# Autodesk Inventor assembly: ASM Printing Head
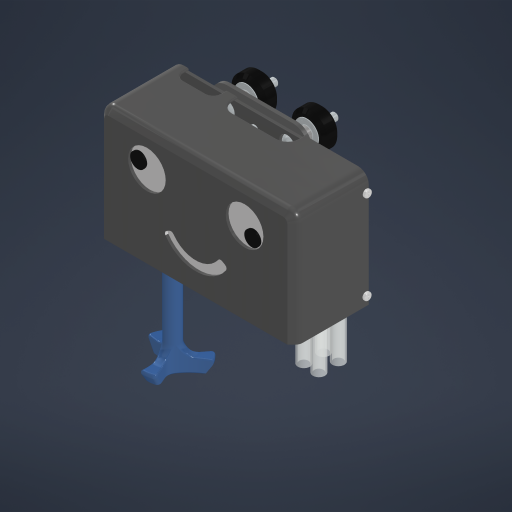
[picture p0: Inventor's stored thumbnail of the model, 512x512]
Saved by Autodesk Inventor 2024 (Build 280153000, 153)
## iProperties
Created: 2018-08-15
Part Number: ASM Printing Head
Document SubType Name: Assembly
Designer: Vincent Larson
Author: Vincent Larson
## Documents named in this file (13)
- C:\Users\Vincent Larson\Downloads\Ender-3 Parts\01 MAIN ASM Ender_3\ASM Printing Head.iam
- C:\Users\Vincent Larson\Downloads\Ender-3 Parts\01 MAIN ASM Ender_3\E plate.ipt
- C:\Users\Vincent Larson\Downloads\Ender-3 Parts\01 MAIN ASM Ender_3\ASM Roller X-Axis.iam
- C:\Users\Vincent Larson\Downloads\Ender-3 Parts\01 MAIN ASM Ender_3\ASM Eccentrical Roller X-Axis.iam
- C:\Users\Vincent Larson\Downloads\Ender-3 Parts\01 MAIN ASM Ender_3\M3X6Pan Head Screw.ipt
- C:\Users\Vincent Larson\Downloads\Motor Bracket.ipt
- C:\Users\Vincent Larson\Downloads\Shaft.ipt
- C:\Users\Vincent Larson\Downloads\Mixing Motor.ipt
- C:\Users\Vincent Larson\Downloads\Tubing.ipt
- C:\Users\Vincent Larson\Downloads\Control Box - Screw.ipt
- C:\Users\Vincent Larson\Downloads\Paper piece.ipt
- C:\Users\Vincent Larson\Downloads\eye.ipt
- C:\Users\Vincent Larson\Downloads\Mixer and nozzle cover.ipt
## Components (24 placed, 12 different names)
1. E plate:1 — Mate:16, Mate:17, Mate:37
2. ASM Roller X-Axis:1 [sub-assembly]
3. ASM Roller X-Axis:2 [sub-assembly]
4. ASM Eccentrical Roller X-Axis:1 [sub-assembly]
5. M3X6Pan Head Screw:1 — Flush:1, Mate:28, Mate:29
6. M3X6Pan Head Screw:2 — Flush:1, Mate:30
7. Motor Bracket:1 — Mate:15, Mate:16, Mate:17, Mate:21, Mate:22, Mate:23, Mate:26, Mate:27, Mate:28, Mate:29, Mate:30, Mate:31, Mate:32, Mate:33, Mate:34, Mate:37, Mate:52, Mate:53
8. Shaft:1 — Mate:55, Mate:56
9. M3X6Pan Head Screw:3 — Flush:4, Mate:22, Flush:5, Flush:6
10. M3X6Pan Head Screw:4 — Flush:4, Mate:15, Mate:23, Flush:6
11. M3X6Pan Head Screw:6 — Mate:21, Flush:5
12. Mixing Motor:1 — Mate:27, Mate:55, Mate:56
13. Tubing:3 — Mate:26, Flush:11, Flush:13
14. Control Box - Screw:1 — Mate:32
15. Control Box - Screw:2 — Mate:31
16. Control Box - Screw:3 — Mate:33
17. Control Box - Screw:4 — Mate:34
18. Tubing:4 — Flush:11, Flush:12
19. Tubing:5 — Flush:12
20. Tubing:6 — Flush:13
21. Paper piece:1 — Mate:50, Mate:51
22. eye:1 — Mate:50
23. eye:2 — Mate:51
24. Mixer and nozzle cover:1 — Mate:52, Mate:53
## Relationships (29: Mate 22, Flush 7)
- Flush:1: M3X6Pan Head Screw:1 ↔ M3X6Pan Head Screw:2
- Flush:4: M3X6Pan Head Screw:3 ↔ M3X6Pan Head Screw:4
- Mate:15: Motor Bracket:1 ↔ M3X6Pan Head Screw:4
- Mate:16: E plate:1 ↔ Motor Bracket:1
- Mate:17: E plate:1 ↔ Motor Bracket:1
- Mate:21: Motor Bracket:1 ↔ M3X6Pan Head Screw:6
- Mate:22: Motor Bracket:1 ↔ M3X6Pan Head Screw:3
- Mate:23: Motor Bracket:1 ↔ M3X6Pan Head Screw:4
- Flush:5: M3X6Pan Head Screw:3 ↔ M3X6Pan Head Screw:6
- Flush:6: M3X6Pan Head Screw:3 ↔ M3X6Pan Head Screw:4
- Mate:26: Motor Bracket:1 ↔ Tubing:3
- Mate:27: Motor Bracket:1 ↔ Mixing Motor:1
- Mate:28: M3X6Pan Head Screw:1 ↔ Motor Bracket:1
- Mate:29: M3X6Pan Head Screw:1 ↔ Motor Bracket:1
- Mate:30: M3X6Pan Head Screw:2 ↔ Motor Bracket:1
- Mate:31: Motor Bracket:1 ↔ Control Box - Screw:2
- Mate:32: Motor Bracket:1 ↔ Control Box - Screw:1
- Mate:33: Motor Bracket:1 ↔ Control Box - Screw:3
- Mate:34: Motor Bracket:1 ↔ Control Box - Screw:4
- Mate:37: E plate:1 ↔ Motor Bracket:1
- Flush:11: Tubing:3 ↔ Tubing:4
- Flush:12: Tubing:4 ↔ Tubing:5
- Flush:13: Tubing:3 ↔ Tubing:6
- Mate:50: Paper piece:1 ↔ eye:1
- Mate:51: Paper piece:1 ↔ eye:2
- Mate:52 (0.5 mm): Motor Bracket:1 ↔ Mixer and nozzle cover:1
- Mate:53: Motor Bracket:1 ↔ Mixer and nozzle cover:1
- Mate:55: Shaft:1 ↔ Mixing Motor:1
- Mate:56: Shaft:1 ↔ Mixing Motor:1
